# Autodesk Inventor assembly: Project
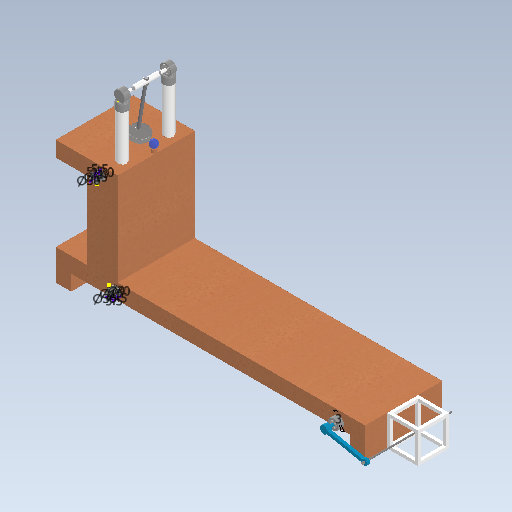
[picture p0: Inventor's stored thumbnail of the model, 512x512]
Saved by Autodesk Inventor 2020 (Build 240168000, 168)
## iProperties
Created: 2021-12-24
Part Number: Project
Document SubType Name: Assembly
Designer: Umur Batuhan Özmen
Author: Umur Batuhan Özmen
## Documents named in this file (19)
- C:\Users\umuro\OneDrive - ikc.edu.tr\Home - Library_Umur\E\Education\2020-2024_Mechatronics\Lessons\MEE203-DINAMIK\Whales_Dynamics_Project\Drawings\Parts\Project.iam
- C:\Users\umuro\OneDrive - ikc.edu.tr\Home - Library_Umur\E\Education\2020-2024_Mechatronics\Lessons\MEE203-DINAMIK\Whales_Dynamics_Project\Drawings\Parts\Marble.ipt
- C:\Users\umuro\OneDrive - ikc.edu.tr\Home - Library_Umur\E\Education\2020-2024_Mechatronics\Lessons\MEE203-DINAMIK\Whales_Dynamics_Project\Drawings\Parts\Platform.ipt
- C:\Users\umuro\OneDrive - ikc.edu.tr\Home - Library_Umur\E\Education\2020-2024_Mechatronics\Lessons\MEE203-DINAMIK\Whales_Dynamics_Project\Drawings\Parts\Rulman_Yatag.ipt
- C:\Users\umuro\OneDrive - ikc.edu.tr\Home - Library_Umur\E\Education\2020-2024_Mechatronics\Lessons\MEE203-DINAMIK\Whales_Dynamics_Project\Drawings\Parts\rulmanyatagıipt.ipt
- C:\Users\umuro\OneDrive - ikc.edu.tr\Home - Library_Umur\E\Education\2020-2024_Mechatronics\Lessons\MEE203-DINAMIK\Whales_Dynamics_Project\Drawings\Parts\Support.ipt
- C:\Users\umuro\OneDrive - ikc.edu.tr\Home - Library_Umur\E\Education\2020-2024_Mechatronics\Lessons\MEE203-DINAMIK\Whales_Dynamics_Project\Drawings\Parts\shaftorj.ipt
- C:\Users\umuro\OneDrive - ikc.edu.tr\Home - Library_Umur\E\Education\2020-2024_Mechatronics\Lessons\MEE203-DINAMIK\Whales_Dynamics_Project\Drawings\Parts\shaftucu2.ipt
- C:\Users\umuro\OneDrive - ikc.edu.tr\Home - Library_Umur\E\Education\2020-2024_Mechatronics\Lessons\MEE203-DINAMIK\Whales_Dynamics_Project\Drawings\Project\Design Accelerator\Bearing1.iam
- C:\Users\umuro\OneDrive - ikc.edu.tr\Home - Library_Umur\E\Education\2020-2024_Mechatronics\Lessons\MEE203-DINAMIK\Whales_Dynamics_Project\Drawings\Parts\Hollow_Cube.ipt
- C:\Users\umuro\OneDrive - ikc.edu.tr\Home - Library_Umur\E\Education\2020-2024_Mechatronics\Lessons\MEE203-DINAMIK\Whales_Dynamics_Project\Drawings\Parts\Hammer.ipt
- C:\Users\umuro\OneDrive - ikc.edu.tr\Home - Library_Umur\E\Education\2020-2024_Mechatronics\Lessons\MEE203-DINAMIK\Whales_Dynamics_Project\Drawings\Parts\Tij.ipt
- C:\Users\umuro\Documents\Inventor\Content Center Files\R2020\en-US\SS-ISO 4035\ISO 4035 - M8SS-ISO.ipt
- C:\Users\umuro\OneDrive - ikc.edu.tr\Home - Library_Umur\E\Education\2020-2024_Mechatronics\Lessons\MEE203-DINAMIK\Whales_Dynamics_Project\Drawings\Project\Design Accelerator\Bearing2.iam
- C:\Users\umuro\OneDrive - ikc.edu.tr\Home - Library_Umur\E\Education\2020-2024_Mechatronics\Lessons\MEE203-DINAMIK\Whales_Dynamics_Project\Drawings\Parts\Rod.ipt
- C:\Users\umuro\OneDrive - ikc.edu.tr\Home - Library_Umur\E\Education\2020-2024_Mechatronics\Lessons\MEE203-DINAMIK\Whales_Dynamics_Project\Drawings\Parts\rodtij.ipt
- C:\Users\umuro\Documents\Inventor\Content Center Files\R2020\en-US\GB_T 41-2000\Nut GB_T 41 M5.ipt
- C:\Users\umuro\OneDrive - ikc.edu.tr\Home - Library_Umur\E\Education\2020-2024_Mechatronics\Lessons\MEE203-DINAMIK\Whales_Dynamics_Project\Drawings\Parts\Pulley.ipt
- C:\Users\umuro\Documents\Inventor\Content Center Files\R2020\en-US\BS EN 24017\ISO 4017 - M8 x 50BS EN.ipt
## Components (28 placed, 17 different names)
1. Marble:1
2. Platform:1 — Rigid:1, Rigid:2, Mate:3, Mate:10, Mate:11, Rotational:13, Rotational:14, Rigid:10, Rigid:11
3. Rulman_Yatag:1 — Rotational:6, Mate:1, Rigid:5
4. Rulman_Yatag:2 — Rotational:7, Mate:1, Mate:2, Rotational:9
5. rulmanyatagıipt:1 — Mate:10, Mate:11, Rotational:11
6. Support:1 — Rigid:1, Rotational:6
7. Support:2 — Rigid:2, Rotational:7
8. shaftorj:1 — Rigid:4, Mate:2, Rigid:6
9. shaftucu2:1 — Rigid:4, Rotational:8
10. shaftucu2:2 — Rotational:10
11. Bearing:1 [sub-assembly] — Rotational:9, Rotational:10
12. Bearing:2 [sub-assembly] — Rigid:5, Rotational:8
13. Hollow_Cube:1 — Mate:3
14. Hammer:1 — Cylindrical:1, Mate:7, Mate:9
15. Tij:1 — Rigid:6, Mate:4, Mate:5, Mate:6, Cylindrical:1, Mate:8
16. SS ISO 4035 M8:1 — Mate:5
17. SS ISO 4035 M8:2 — Mate:4
18. SS ISO 4035 M8:3 — Mate:8, Mate:9
19. SS ISO 4035 M8:4 — Mate:6, Mate:7
20. Bearing:3 [sub-assembly] — Rotational:11, Rotational:12
21. Rod:1 — Rotational:12, Rigid:7, Rigid:8, Rigid:9
22. rodtij:1 — Rigid:7
23. Nut GB/T 41-2000 M 5:1 — Rigid:8
24. Nut GB/T 41-2000 M 5:2 — Rigid:9
25. Pulley:1 — Rotational:14
26. Pulley:2 — Rotational:13
27. BS EN 24017 - Metric M8 x 50:1 — Rigid:11
28. BS EN 24017 - Metric M8 x 50:2 — Rigid:10
## Relationships (31: Mate 11, WeldJoint 10, RevoluteJoint 9, CylindricalJoint 1)
- Rigid:1 [WeldJoint]: Platform:1 ↔ Support:1
- Rigid:2 [WeldJoint]: Platform:1 ↔ Support:2
- Rigid:4 [WeldJoint] (-6 mm): shaftorj:1 ↔ shaftucu2:1
- Rotational:6 [RevoluteJoint]: Rulman_Yatag:1 ↔ Support:1
- Rotational:7 [RevoluteJoint]: Rulman_Yatag:2 ↔ Support:2
- Mate:1: Rulman_Yatag:1 ↔ Rulman_Yatag:2
- Mate:2: Rulman_Yatag:2 ↔ shaftorj:1
- Rigid:5 [WeldJoint]: Rulman_Yatag:1 ↔ Bearing:2
- Rotational:8 [RevoluteJoint] (-5 mm): shaftucu2:1 ↔ Bearing:2
- Rotational:9 [RevoluteJoint]: Rulman_Yatag:2 ↔ Bearing:1
- Rotational:10 [RevoluteJoint] (3 mm): shaftucu2:2 ↔ Bearing:1
- Mate:3: Platform:1 ↔ Hollow_Cube:1
- Rigid:6 [WeldJoint] (3 mm): shaftorj:1 ↔ Tij:1
- Mate:4: Tij:1 ↔ SS ISO 4035 M8:2
- Mate:5: Tij:1 ↔ SS ISO 4035 M8:1
- Mate:6: Tij:1 ↔ SS ISO 4035 M8:4
- Cylindrical:1: Hammer:1 ↔ Tij:1
- Mate:7: Hammer:1 ↔ SS ISO 4035 M8:4
- Mate:8: Tij:1 ↔ SS ISO 4035 M8:3
- Mate:9: Hammer:1 ↔ SS ISO 4035 M8:3
- Mate:10: Platform:1 ↔ rulmanyatagıipt:1
- Mate:11: Platform:1 ↔ rulmanyatagıipt:1
- Rotational:11 [RevoluteJoint] (-3 mm): rulmanyatagıipt:1 ↔ Bearing:3
- Rotational:12 [RevoluteJoint] (-1.95 mm): Bearing:3 ↔ Rod:1
- Rigid:7 [WeldJoint] (-6 mm): Rod:1 ↔ rodtij:1
- Rigid:8 [WeldJoint]: Rod:1 ↔ Nut GB/T 41-2000 M 5:1
- Rigid:9 [WeldJoint]: Rod:1 ↔ Nut GB/T 41-2000 M 5:2
- Rotational:13 [RevoluteJoint] (-5 mm): Platform:1 ↔ Pulley:2
- Rotational:14 [RevoluteJoint] (-5 mm): Platform:1 ↔ Pulley:1
- Rigid:10 [WeldJoint]: Platform:1 ↔ BS EN 24017 - Metric M8 x 50:2
- Rigid:11 [WeldJoint]: Platform:1 ↔ BS EN 24017 - Metric M8 x 50:1
